# Autodesk Inventor assembly: bat_mount_b
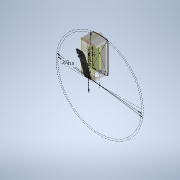
[picture p0: Inventor's stored thumbnail of the model, 180x180]
Saved by Autodesk Inventor 2020 (Build 240168000, 168)
## iProperties
Created: 2024-02-12
Part Number: bat_mount_b
Document SubType Name: Assembly
Designer: 4s
Author: 4s
## Documents named in this file (3)
- C:\Users\4s\Documents\Inventor models\Asterisk\robot_v2\bat_mount_b.iam
- C:\Users\4s\Documents\Inventor models\Asterisk\robot_v2\bat_mount003.ipt
- C:\Users\4s\Documents\Inventor models\Asterisk\bat_lock02.ipt
## Components (2 placed, 2 different names)
1. bat_mount003:1 — Совмещение:1, Совмещение:2, Совмещение:3, Совмещение:4, Заподлицо:1
2. bat_lock02:1 — Совмещение:1, Совмещение:2, Заподлицо:1
## Relationships (5: Mate 4, Flush 1)
- Совмещение:1 [Mate] (-4.5 mm): bat_mount003:1 ↔ bat_lock02:1
- Совмещение:2 [Mate] (7.5 mm): bat_mount003:1 ↔ bat_lock02:1
- Совмещение:3 [Mate]: bat_mount003:1
- Совмещение:4 [Mate]: bat_mount003:1
- Заподлицо:1 [Flush]: bat_mount003:1 ↔ bat_lock02:1
